# Autodesk Inventor assembly: Toughbox-mini_MIR7_MIR
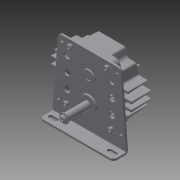
[picture p0: Inventor's stored thumbnail of the model, 180x180]
Saved by Autodesk Inventor 2015 (Build 190159000, 159)
## iProperties
Created: 2015-01-11
Part Number: Toughbox-mini_MIR7_MIR
Document SubType Name: Assembly
Designer: whitaus15
Author: whitaus15
Author: Unknown
Title: S:/Products/Gearboxes Spur Single Stage/Toughbox/Toughbox Mini/Toughbox-Mini.stp
Organization: Unknown
Description: Unknown
Sending System: Unknown
Preprocessor: XStep 1.0
## Documents named in this file (19)
- \\lhssvr02\Homedirs\Robotics Club\CAD Model 2015\Parts Folder\Gear Boxes\Toughbox-mini_MIR7_MIR.iam
- \\lhssvr02\Homedirs\Robotics Club\CAD Model 2015\Parts Folder\Gear Boxes\Imported Components\Toughbox-mini\r6zz_MIR7_MIR.ipt
- \\lhssvr02\Homedirs\Robotics Club\CAD Model 2015\Parts Folder\Gear Boxes\Imported Components\Toughbox-mini\Toughbox_d03_MIR7_MIR.ipt
- \\lhssvr02\Homedirs\Robotics Club\CAD Model 2015\Parts Folder\Gear Boxes\Imported Components\Toughbox-mini\Toughbox_d07_MIR7_MIR.ipt
- \\lhssvr02\Homedirs\Robotics Club\CAD Model 2015\Parts Folder\Gear Boxes\Imported Components\Toughbox-mini\Toughbox_d05_MIR7_MIR.ipt
- \\lhssvr02\Homedirs\Robotics Club\CAD Model 2015\Parts Folder\Gear Boxes\Imported Components\Toughbox-mini\Toughbox_d08_MIR7_MIR.ipt
- \\lhssvr02\Homedirs\Robotics Club\CAD Model 2015\Parts Folder\Gear Boxes\Imported Components\Toughbox-mini\Toughbox_d06_MIR7_MIR.ipt
- \\lhssvr02\Homedirs\Robotics Club\CAD Model 2015\Parts Folder\Gear Boxes\Imported Components\Toughbox-mini\fr-6-zz_MIR7_MIR.ipt
- \\lhssvr02\Homedirs\Robotics Club\CAD Model 2015\Parts Folder\Gear Boxes\Imported Components\Toughbox-mini\fr-8-zz_MIR7_MIR.ipt
- \\lhssvr02\Homedirs\Robotics Club\CAD Model 2015\Parts Folder\Gear Boxes\Imported Components\Toughbox-mini\10-32_nylock_nut_MIR7_MIR.ipt
- \\lhssvr02\Homedirs\Robotics Club\CAD Model 2015\Parts Folder\Gear Boxes\Imported Components\Toughbox-mini\5-16_washer_MIR7_MIR.ipt
- \\lhssvr02\Homedirs\Robotics Club\CAD Model 2015\Parts Folder\Gear Boxes\Imported Components\Toughbox-mini\Toughbox_d09_MIR7_MIR.ipt
- \\lhssvr02\Homedirs\Robotics Club\CAD Model 2015\Parts Folder\Gear Boxes\Imported Components\Toughbox-mini\8mm_spring_clip_MIR7_MIR.ipt
- \\lhssvr02\Homedirs\Robotics Club\CAD Model 2015\Parts Folder\Gear Boxes\Imported Components\Toughbox-mini\Toughbox-mini_d01-5-12_MIR7_MIR.ipt
- \\lhssvr02\Homedirs\Robotics Club\CAD Model 2015\Parts Folder\Gear Boxes\Imported Components\Toughbox-mini\Toughbox-mini_d02_MIR7_MIR.ipt
- \\lhssvr02\Homedirs\Robotics Club\CAD Model 2015\Parts Folder\Gear Boxes\Imported Components\Toughbox-mini\250_washer_MIR7_MIR.ipt
- \\lhssvr02\Homedirs\Robotics Club\CAD Model 2015\Parts Folder\Gear Boxes\Imported Components\Toughbox-mini\14-20x0500_bhcs_MIR7_MIR.ipt
- \\lhssvr02\Homedirs\Robotics Club\CAD Model 2015\Parts Folder\Gear Boxes\Imported Components\Toughbox-mini\125x124x700_key_MIR7_MIR.ipt
- \\lhssvr02\Homedirs\Robotics Club\CAD Model 2015\Parts Folder\Gear Boxes\Imported Components\Toughbox-mini\10-32x0625_shcs_MIR7_MIR.ipt
## Components (34 placed, 18 different names)
1. r6zz_MIR7_MIR:1
2. r6zz_MIR7_MIR:2
3. Toughbox_d03_MIR7_MIR:1
4. Toughbox_d07_MIR7_MIR:1
5. Toughbox_d05_MIR7_MIR:1
6. Toughbox_d08_MIR7_MIR:1
7. Toughbox_d06_MIR7_MIR:1
8. fr-6-zz_MIR7_MIR:1
9. fr-8-zz_MIR7_MIR:1
10. 10-32_nylock_nut_MIR7_MIR:1
11. 10-32_nylock_nut_MIR7_MIR:2
12. 10-32_nylock_nut_MIR7_MIR:3
13. 10-32_nylock_nut_MIR7_MIR:4
14. 5-16_washer_MIR7_MIR:1
15. 5-16_washer_MIR7_MIR:2
16. 5-16_washer_MIR7_MIR:3
17. 5-16_washer_MIR7_MIR:4
18. Toughbox_d09_MIR7_MIR:1
19. Toughbox_d09_MIR7_MIR:2
20. 8mm_spring_clip_MIR7_MIR:1
21. 8mm_spring_clip_MIR7_MIR:2
22. Toughbox-mini_d01-5-12_MIR7_MIR:1 — Mate:1
23. Toughbox-mini_d02_MIR7_MIR:1 — Mate:1, Insert:1, Insert:2
24. 250_washer_MIR7_MIR:1
25. 14-20x0500_bhcs_MIR7_MIR:1
26. 125x124x700_key_MIR7_MIR:1
27. 10-32x0625_shcs_MIR7_MIR:1
28. 10-32x0625_shcs_MIR7_MIR:2
29. 10-32x0625_shcs_MIR7_MIR:3 — Insert:1
30. 10-32x0625_shcs_MIR7_MIR:4
31. 10-32x0625_shcs_MIR7_MIR:5 — Insert:2
32. 10-32x0625_shcs_MIR7_MIR:6
33. 10-32x0625_shcs_MIR7_MIR:7
34. 10-32x0625_shcs_MIR7_MIR:8
## Relationships (3: Insert 2, Mate 1)
- Mate:1: Toughbox-mini_d01-5-12_MIR7_MIR:1 ↔ Toughbox-mini_d02_MIR7_MIR:1
- Insert:1: Toughbox-mini_d02_MIR7_MIR:1 ↔ 10-32x0625_shcs_MIR7_MIR:3
- Insert:2: Toughbox-mini_d02_MIR7_MIR:1 ↔ 10-32x0625_shcs_MIR7_MIR:5
